# Autodesk Inventor assembly: Articuled-Robot
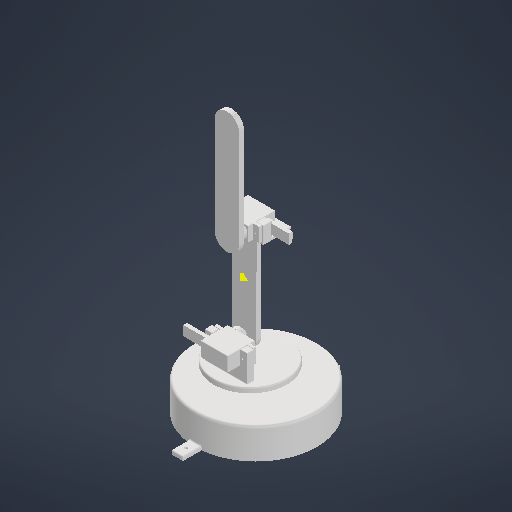
[picture p0: Inventor's stored thumbnail of the model, 512x512]
Saved by Autodesk Inventor 2026 (Build 300175000, 175)
## iProperties
Created: 2026-02-13
Part Number: Articuled-Robot
Document SubType Name: Assembly
Designer: Jakob Dorninger
Author: Jakob Dorninger
## Documents named in this file (6)
- C:\05_Projekte\Articulated-Robot\CAD\Articuled-Robot.iam
- C:\05_Projekte\Articulated-Robot\CAD\Base.ipt
- C:\05_Projekte\Articulated-Robot\CAD\Motor.ipt
- C:\05_Projekte\Articulated-Robot\CAD\Shoulder.ipt
- C:\05_Projekte\Articulated-Robot\CAD\L1.ipt
- C:\05_Projekte\Articulated-Robot\CAD\L2.ipt
## Components (7 placed, 5 different names)
1. Base:1 — Passend:1, Passend:3, Passend:17
2. Motor:1 — Passend:1, Passend:3, Passend:4, Passend:5, Passend:17
3. Shoulder:1 — Passend:4, Passend:5, Winkel:1, Passend:6, Passend:8, Passend:9
4. Motor:2 — Passend:6, Passend:8, Passend:9, Passend:10, Passend:11
5. L1:1 — Passend:10, Passend:11, Passend:12, Passend:13, Passend:14
6. Motor:3 — Passend:12, Passend:13, Passend:14, Passend:15, Passend:16
7. L2:1 — Passend:15, Passend:16
## Relationships (16: Mate 15, Angle 1)
- Passend:1 [Mate] (1.25 mm): Base:1 ↔ Motor:1
- Passend:3 [Mate] (0.25 mm): Base:1 ↔ Motor:1
- Passend:4 [Mate]: Motor:1 ↔ Shoulder:1
- Passend:5 [Mate]: Motor:1 ↔ Shoulder:1
- Winkel:1 [Angle] (0 deg): Shoulder:1
- Passend:6 [Mate]: Shoulder:1 ↔ Motor:2
- Passend:8 [Mate]: Shoulder:1 ↔ Motor:2
- Passend:9 [Mate]: Shoulder:1 ↔ Motor:2
- Passend:10 [Mate]: Motor:2 ↔ L1:1
- Passend:11 [Mate]: Motor:2 ↔ L1:1
- Passend:12 [Mate]: L1:1 ↔ Motor:3
- Passend:13 [Mate]: L1:1 ↔ Motor:3
- Passend:14 [Mate]: L1:1 ↔ Motor:3
- Passend:15 [Mate]: Motor:3 ↔ L2:1
- Passend:16 [Mate]: Motor:3 ↔ L2:1
- Passend:17 [Mate]: Base:1 ↔ Motor:1
